# Autodesk Inventor assembly: Brazo Robótivo 2023 v144
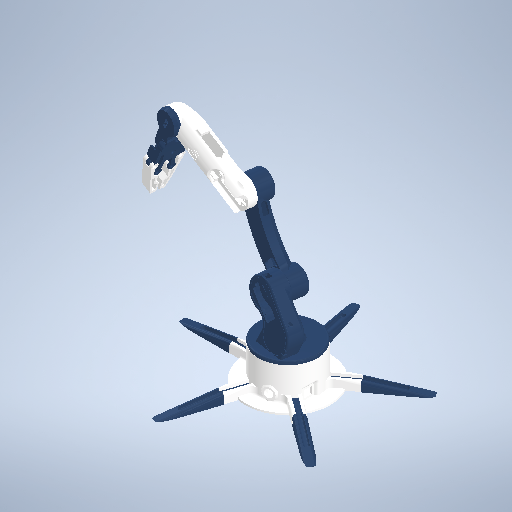
[picture p0: Inventor's stored thumbnail of the model, 512x512]
Saved by Autodesk Inventor 2026 (Build 300175000, 175)
## iProperties
Created: 2024-04-02
Part Number: Brazo Robótivo 2023 v144
Document SubType Name: Assembly
Designer: Gustavo Sousa
Sending System: Autodesk Translation Framework v12.20.1.177
Preprocessor: ST-DEVELOPER v20
Title: Brazo Robtivo 2023 v144.step
## Documents named in this file (22)
- C:\Users\carlo\Documents\Projeto - Braco Robotico\Design\braco_robotico\Brazo Robótivo 2023 v144.iam
- C:\Users\carlo\Documents\Projeto - Braco Robotico\Design\braco_robotico\Brazo Robótivo 2023 v144\Engranaje1.ipt
- C:\Users\carlo\Documents\Projeto - Braco Robotico\Design\braco_robotico\Brazo Robótivo 2023 v144\Engranaje2.ipt
- C:\Users\carlo\Documents\Projeto - Braco Robotico\Design\braco_robotico\Brazo Robótivo 2023 v144\Barra2.ipt
- C:\Users\carlo\Documents\Projeto - Braco Robotico\Design\braco_robotico\Brazo Robótivo 2023 v144\Barra1.ipt
- C:\Users\carlo\Documents\Projeto - Braco Robotico\Design\braco_robotico\Brazo Robótivo 2023 v144\Pinza1.ipt
- C:\Users\carlo\Documents\Projeto - Braco Robotico\Design\braco_robotico\Brazo Robótivo 2023 v144\Pinza2.ipt
- C:\Users\carlo\Documents\Projeto - Braco Robotico\Design\braco_robotico\Brazo Robótivo 2023 v144\Base de la garra.ipt
- C:\Users\carlo\Documents\Projeto - Braco Robotico\Design\braco_robotico\Brazo Robótivo 2023 v144\Base (1) (1).ipt
- C:\Users\carlo\Documents\Projeto - Braco Robotico\Design\braco_robotico\Brazo Robótivo 2023 v144\Antebrazo (4).ipt
- C:\Users\carlo\Documents\Projeto - Braco Robotico\Design\braco_robotico\Brazo Robótivo 2023 v144\Muñeca.ipt
- C:\Users\carlo\Documents\Projeto - Braco Robotico\Design\braco_robotico\Brazo Robótivo 2023 v144\Eje Central.ipt
- C:\Users\carlo\Documents\Projeto - Braco Robotico\Design\braco_robotico\Brazo Robótivo 2023 v144\Tapa Eje.ipt
- C:\Users\carlo\Documents\Projeto - Braco Robotico\Design\braco_robotico\Brazo Robótivo 2023 v144\Tapa Base.ipt
- C:\Users\carlo\Documents\Projeto - Braco Robotico\Design\braco_robotico\Brazo Robótivo 2023 v144\Brazo.ipt
- C:\Users\carlo\Documents\Projeto - Braco Robotico\Design\braco_robotico\Brazo Robótivo 2023 v144\Tapa garra.ipt
- C:\Users\carlo\Documents\Projeto - Braco Robotico\Design\braco_robotico\Brazo Robótivo 2023 v144\Pata1.ipt
- C:\Users\carlo\Documents\Projeto - Braco Robotico\Design\braco_robotico\Brazo Robótivo 2023 v144\Pata2.ipt
- C:\Users\carlo\Documents\Projeto - Braco Robotico\Design\braco_robotico\Brazo Robótivo 2023 v144\Pata3.ipt
- C:\Users\carlo\Documents\Projeto - Braco Robotico\Design\braco_robotico\Brazo Robótivo 2023 v144\Pata4.ipt
- C:\Users\carlo\Documents\Projeto - Braco Robotico\Design\braco_robotico\Brazo Robótivo 2023 v144\Pata5.ipt
- C:\Users\carlo\Documents\Projeto - Braco Robotico\Design\braco_robotico\Brazo Robótivo 2023 v144\Seguro de servomotor.ipt
## Components (21 placed, 21 different names)
1. Engranaje1:1 — Mate:24, Mate:25, Insert:10
2. Engranaje2:1 — Mate:22, Mate:23, Insert:11
3. Barra2:1 — Insert:8, Mate:27
4. Barra1:1 — Insert:9, Mate:26
5. Pinza1:1 — Insert:10, Mate:26
6. Pinza2:1 — Insert:11, Mate:27
7. Base de la garra:1 — Insert:6, Mate:21, Insert:8, Insert:9, Insert:12
8. Base (1) (1):1 — Mate:7, Mate:8, Mate:9, Mate:10, Mate:11, Mate:12, Mate:13, Mate:14, Mate:15, Mate:16, Mate:17, Mate:18, Insert:1
9. Antebrazo (4):1 — Insert:2, Insert:4
10. Muñeca:1 — Insert:5, Insert:12
11. Eje Central:1 — Insert:1, Mate:19, Mate:20, Insert:2
12. Tapa Eje:1 — Mate:19, Mate:20
13. Tapa Base:1 — Mate:17, Mate:18
14. Brazo:1 — Insert:3, Insert:4, Insert:5
15. Tapa garra:1 — Insert:6, Mate:21, Mate:22, Mate:23, Mate:24, Mate:25
16. Pata1:1 — Mate:9, Mate:10
17. Pata2:1 — Mate:11, Mate:12
18. Pata3:1 — Mate:15, Mate:16
19. Pata4:1 — Mate:13, Mate:14
20. Pata5:1 — Mate:7, Mate:8
21. Seguro de servomotor:1 — Insert:3
## Relationships (32: Mate 21, Insert 11)
- Mate:7: Base (1) (1):1 ↔ Pata5:1
- Mate:8: Base (1) (1):1 ↔ Pata5:1
- Mate:9: Base (1) (1):1 ↔ Pata1:1
- Mate:10: Base (1) (1):1 ↔ Pata1:1
- Mate:11: Base (1) (1):1 ↔ Pata2:1
- Mate:12: Base (1) (1):1 ↔ Pata2:1
- Mate:13: Base (1) (1):1 ↔ Pata4:1
- Mate:14: Base (1) (1):1 ↔ Pata4:1
- Mate:15: Base (1) (1):1 ↔ Pata3:1
- Mate:16: Base (1) (1):1 ↔ Pata3:1
- Mate:17: Base (1) (1):1 ↔ Tapa Base:1
- Mate:18: Base (1) (1):1 ↔ Tapa Base:1
- Insert:1: Base (1) (1):1 ↔ Eje Central:1
- Mate:19: Eje Central:1 ↔ Tapa Eje:1
- Mate:20 (1.05 mm): Eje Central:1 ↔ Tapa Eje:1
- Insert:2: Antebrazo (4):1 ↔ Eje Central:1
- Insert:3: Brazo:1 ↔ Seguro de servomotor:1
- Insert:4: Antebrazo (4):1 ↔ Brazo:1
- Insert:5: Muñeca:1 ↔ Brazo:1
- Insert:6: Base de la garra:1 ↔ Tapa garra:1
- Mate:21: Base de la garra:1 ↔ Tapa garra:1
- Insert:8: Barra2:1 ↔ Base de la garra:1
- Insert:9: Barra1:1 ↔ Base de la garra:1
- Mate:22: Engranaje2:1 ↔ Tapa garra:1
- Mate:23: Engranaje2:1 ↔ Tapa garra:1
- Mate:24: Engranaje1:1 ↔ Tapa garra:1
- Mate:25: Engranaje1:1 ↔ Tapa garra:1
- Insert:10 (0.5 mm): Engranaje1:1 ↔ Pinza1:1
- Mate:26: Barra1:1 ↔ Pinza1:1
- Insert:11: Engranaje2:1 ↔ Pinza2:1
- Mate:27: Barra2:1 ↔ Pinza2:1
- Insert:12: Base de la garra:1 ↔ Muñeca:1
